# Autodesk Inventor assembly: outer
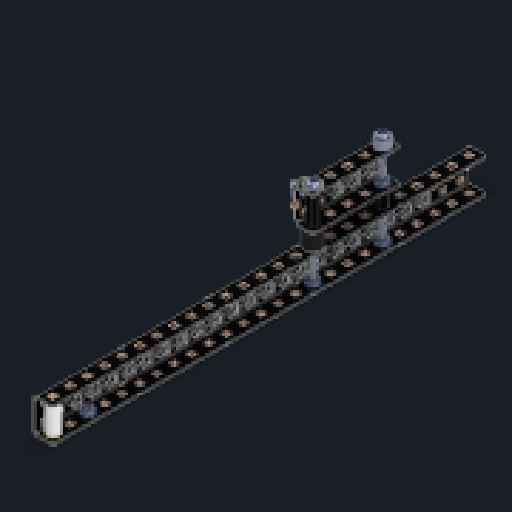
[picture p0: Inventor's stored thumbnail of the model, 512x512]
Saved by Autodesk Inventor 2024 (Build 280153000, 153)
## iProperties
Created: 2024-03-01
Part Number: outer
Document SubType Name: Assembly
Designer: Averey Ku
Author: Averey Ku
## Documents named in this file (22)
- D:\vex_robotics\hardware\cad\smolbot\chassis\drivebay\outer.iam
- D:\vex_robotics\hardware\cad\VEX-CAD-Inventor-1.41\Structure\C Channel\Aluminum 1x2x1\Alu C 1x2x1x25.ipt
- D:\vex_robotics\hardware\cad\VEX-CAD-Inventor-1.41\Motion\Shaft LS\Bearing Flat Low Profile.ipt
- D:\vex_robotics\hardware\cad\hardware\.375 OD Aluminum Spacer 0.875.ipt
- D:\vex_robotics\hardware\cad\VEX-CAD-Inventor-1.41\Structure\Hardware\Nut Keps.ipt
- D:\vex_robotics\hardware\cad\VEX-CAD-Inventor-1.41\Structure\Hardware\Screw Steel - Star\SScrew Star Smooth 1.250.ipt
- D:\vex_robotics\hardware\cad\VEX-CAD-Inventor-1.41\Structure\Hardware\Screw Steel - Star.ipt
- D:\vex_robotics\hardware\cad\VEX-CAD-Inventor-1.41\Structure\Standoff\Standoff .50.ipt
- D:\vex_robotics\hardware\cad\VEX-CAD-Inventor-1.41\Structure\Standoff.ipt
- D:\vex_robotics\hardware\cad\VEX-CAD-Inventor-1.41\Structure\C Channel\Aluminum 1x2x1\Alu C 1x2x1x5.ipt
- D:\vex_robotics\hardware\cad\VEX-CAD-Inventor-1.41\Motion\Spacers\Spacer Nylon .500 OD\NSpacer Black .500 OD x .500.ipt
- D:\vex_robotics\hardware\cad\VEX-CAD-Inventor-1.41\Motion\Spacers\Spacer Nylon .500 OD.ipt
- D:\vex_robotics\hardware\cad\VEX-CAD-Inventor-1.41\Structure\Hardware\Screw Steel - Star\SScrew Star Smooth 1.750.ipt
- D:\vex_robotics\hardware\cad\VEX-CAD-Inventor-1.41\Structure\Standoff\Standoff .875.ipt
- D:\vex_robotics\hardware\cad\VEX-CAD-Inventor-1.41\Structure\Hardware\Screw Shoulder Robosource\SScrew Shoulder Smooth .290 x .09.ipt
- D:\vex_robotics\hardware\cad\VEX-CAD-Inventor-1.41\Structure\Hardware\Screw Shoulder Robosource.ipt
- D:\vex_robotics\hardware\cad\VEX-CAD-Inventor-1.41\Motion\Spacers\Washer Teflon\TWasher .500 OD x .04000.ipt
- D:\vex_robotics\hardware\cad\VEX-CAD-Inventor-1.41\Motion\Spacers\Washer Teflon.ipt
- D:\vex_robotics\hardware\cad\VEX-CAD-Inventor-1.41\Structure\Hardware\Screw Steel - Star\SScrew Star Smooth .375.ipt
- D:\vex_robotics\hardware\cad\VEX-CAD-Inventor-1.41\Motion\Spacers\Washer Delrin\DWasher .500 OD x .062500.ipt
- D:\vex_robotics\hardware\cad\VEX-CAD-Inventor-1.41\Motion\Shaft LS\Shaft Collar ipts\Shaft Collar No Screw.ipt
- D:\vex_robotics\hardware\cad\VEX-CAD-Inventor-1.41\Structure\Hardware\Screw Steel - Star\SScrew Star Smooth 1.500.ipt
## Components (30 placed, 16 different names)
1. Alu C 1x2x1x25:1 — Insert:1, Mate:1, Insert:2, Mate:2, Insert:3, Mate:3, Insert:4, Mate:4, Insert:5, Mate:5, Insert:6, Mate:6, Insert:7, Mate:7, Insert:8, Insert:9, Insert:10, Insert:20, Insert:21, Insert:36, Insert:37, Insert:38, Insert:40, Insert:43, Insert:44
2. Bearing Flat Low Profile:1 — Insert:1, Mate:1
3. Bearing Flat Low Profile:2 — Insert:2, Mate:2
4. Bearing Flat Low Profile:3 — Insert:3, Mate:3
5. Bearing Flat Low Profile:4 — Insert:4, Mate:4
6. Bearing Flat Low Profile:5 — Insert:7, Mate:7
7. Bearing Flat Low Profile:6 — Insert:6, Mate:6
8. Bearing Flat Low Profile:7 — Insert:5, Mate:5
9. .375 OD Aluminum Spacer 0.875:1 — Insert:8
10. Nut Keps:1 — Insert:10
11. Nut Keps:2 — Insert:9
12. Nut Keps:3 — Insert:37
13. Nut Keps:4 — Insert:36
14. Nut Keps:5 — Insert:21
15. Nut Keps:6 — Insert:20
16. Bearing Flat Low Profile:8 — Insert:34, Mate:9
17. Alu C 1x2x1x5:1 — Insert:34, Mate:9, Insert:42, Insert:46, Insert:48, Insert:50, Insert:51, Insert:52, Insert:53, Angle:1, Mate:10, Mate:11, Insert:55
18. NSpacer Black .500 OD x .500:1 — Insert:38, Mate:10
19. SScrew Star Smooth 1.750:3 — Insert:40
20. Standoff .875:1 — Insert:42
21. Standoff .50:2 — Insert:44, Mate:11, Insert:55
22. SScrew Star Smooth 1.250:4 — Insert:43
23. Nut Keps:7 — Insert:46
24. SScrew Shoulder Smooth .290 x .09:1 — Insert:49
25. TWasher .500 OD x .04000:1 — Insert:48, Insert:49
26. SScrew Star Smooth .375:6 — Insert:50
27. DWasher .500 OD x .062500:1 — Insert:51
28. Nut Keps:8 — Insert:52
29. Shaft Collar No Screw:1 — Insert:53, Angle:1, Insert:54
30. SScrew Star Smooth 1.500:7 — Insert:54
## Relationships (40: Insert 29, Mate 10, Angle 1)
- Insert:1: Alu C 1x2x1x25:1 ↔ Bearing Flat Low Profile:1
- Mate:1: Alu C 1x2x1x25:1 ↔ Bearing Flat Low Profile:1
- Insert:2: Alu C 1x2x1x25:1 ↔ Bearing Flat Low Profile:2
- Mate:2: Alu C 1x2x1x25:1 ↔ Bearing Flat Low Profile:2
- Insert:3: Alu C 1x2x1x25:1 ↔ Bearing Flat Low Profile:3
- Mate:3: Alu C 1x2x1x25:1 ↔ Bearing Flat Low Profile:3
- Insert:4: Alu C 1x2x1x25:1 ↔ Bearing Flat Low Profile:4
- Mate:4: Alu C 1x2x1x25:1 ↔ Bearing Flat Low Profile:4
- Insert:5: Alu C 1x2x1x25:1 ↔ Bearing Flat Low Profile:7
- Mate:5: Alu C 1x2x1x25:1 ↔ Bearing Flat Low Profile:7
- Insert:6: Alu C 1x2x1x25:1 ↔ Bearing Flat Low Profile:6
- Mate:6: Alu C 1x2x1x25:1 ↔ Bearing Flat Low Profile:6
- Insert:7: Alu C 1x2x1x25:1 ↔ Bearing Flat Low Profile:5
- Mate:7: Alu C 1x2x1x25:1 ↔ Bearing Flat Low Profile:5
- Insert:8: Alu C 1x2x1x25:1 ↔ .375 OD Aluminum Spacer 0.875:1
- Insert:9: Alu C 1x2x1x25:1 ↔ Nut Keps:2
- Insert:10: Alu C 1x2x1x25:1 ↔ Nut Keps:1
- Insert:20: Alu C 1x2x1x25:1 ↔ Nut Keps:6
- Insert:21: Alu C 1x2x1x25:1 ↔ Nut Keps:5
- Insert:34: Bearing Flat Low Profile:8 ↔ Alu C 1x2x1x5:1
- Mate:9: Bearing Flat Low Profile:8 ↔ Alu C 1x2x1x5:1
- Insert:36: Alu C 1x2x1x25:1 ↔ Nut Keps:4
- Insert:37: Alu C 1x2x1x25:1 ↔ Nut Keps:3
- Insert:38: Alu C 1x2x1x25:1 ↔ NSpacer Black .500 OD x .500:1
- Insert:40: Alu C 1x2x1x25:1 ↔ SScrew Star Smooth 1.750:3
- Insert:42: Alu C 1x2x1x5:1 ↔ Standoff .875:1
- Insert:43: Alu C 1x2x1x25:1 ↔ SScrew Star Smooth 1.250:4
- Insert:44: Alu C 1x2x1x25:1 ↔ Standoff .50:2
- Insert:46: Alu C 1x2x1x5:1 ↔ Nut Keps:7
- Insert:48: Alu C 1x2x1x5:1 ↔ TWasher .500 OD x .04000:1
- Insert:49: SScrew Shoulder Smooth .290 x .09:1 ↔ TWasher .500 OD x .04000:1
- Insert:50: Alu C 1x2x1x5:1 ↔ SScrew Star Smooth .375:6
- Insert:51: Alu C 1x2x1x5:1 ↔ DWasher .500 OD x .062500:1
- Insert:52: Alu C 1x2x1x5:1 ↔ Nut Keps:8
- Insert:53: Alu C 1x2x1x5:1 ↔ Shaft Collar No Screw:1
- Angle:1 (0 deg): Alu C 1x2x1x5:1 ↔ Shaft Collar No Screw:1
- Insert:54: Shaft Collar No Screw:1 ↔ SScrew Star Smooth 1.500:7
- Mate:10: Alu C 1x2x1x5:1 ↔ NSpacer Black .500 OD x .500:1
- Mate:11: Alu C 1x2x1x5:1 ↔ Standoff .50:2
- Insert:55: Alu C 1x2x1x5:1 ↔ Standoff .50:2
